# Autodesk Inventor assembly: FO-022
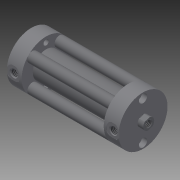
[picture p0: Inventor's stored thumbnail of the model, 180x180]
Saved by Autodesk Inventor 2014 (Build 180170000, 170)
## iProperties
Category: PARTsolutions
Company: BIMBA
Created: 2014-01-19
Part Number: FO-022
Catalog Web Link: www.cadenas.de
Description: FO, FOD, FOR, FOS-Bimba FLAT-1
Vendor: BIMBA
Document SubType Name: Assembly
Designer: Andrew Toennies
Manufacturer: BIMBA
PSOL_IDENT_0: {$CADENAS_DATA\23d-libs\bimba\bimba\bimba_imperial\bimba_full_line\flat_cylinders\fo1\fo1_asmtab.prj
PSOL_IDENT_1: },275 {VTYP=3D},{STYP=ASSTAB},{NB=FO-022},{LINA=FO-022},{NN=FO, FOD, FOR, FOS},{DATE=11.10.2013 12:3
PSOL_IDENT_2: 5:34},{GEOMDATE=17.11.2012 07:08:13},{VERSION=},{LINEID=10},{LINESUBID=-1},{WBVAR=STROKE,ACTING,MNTR
PSOL_IDENT_3: ,MNTF,EE,EEL,B,RT,G,HR,HD,FO,FS,M,PP,TO,S,STPT1,STPT2,STPT3,STPT4,W,Y,RP,CB,TB}  {NB=FO-022},{LINA=F
PSOL_IDENT_4: O-022},{KT=DUMMY},{PN=FO-022},{PNA=(NO ACCESSORIES)},{PNC=FO-022},{BORE=9/16\" (02)},{BORE1=0.562500
PSOL_IDENT_5: 00},{BOREPN=02},{STROKE=2},{STROKEMAX=10.00000000},{ACTING=},{ACTINGALG='','Double Acting, Single En
PSOL_IDENT_6: d Rod [FO]', 'D'  , 'Double Acting, Double End Rod [FOD]', 'R', 'Reverse Acting [FOR]', 'S'  ,'Singl
PSOL_IDENT_7: e Acting [FOS]'},{MNTR=},{MNTF=},{MNT=},{MNTALG='','Standard Counterbored Mounting Holes','1','Pivot
PSOL_IDENT_8: Mount','1N','Pivot Mount 90 Deg. from Standard','3','Threaded Mounting Holes, Both Ends','3F','Thre
PSOL_IDENT_9: aded Mounting Holes, Front','3R','Threaded Mounting Holes, Rear','4','Screw Clearance Holes, Both En
PSOL_IDENT_10: ds','4F','Screw Clearance Holes, Front','4R','Screw Clearance Holes, Rear','5','Nose Mount'},{EEMAX=
PSOL_IDENT_11: 8},{EE=},{EEALG='','Without Extra Extension','EE','With Extra Extension'},{EEL=0.000},{EELALG=0},{B=
PSOL_IDENT_12: },{BALG='','Without Bumper','B','Bumper, Both Ends','BR','Bumper, Rear Only','BF','Bumper, Front Onl
PSOL_IDENT_13: y'},{RT=},{RTALG='', 'Standard Female Thread #8-32',  'MT', 'Male Rod End (Fine) #8-32 [MT]', 'NT'
PSOL_IDENT_14: , 'Non-Threaded Rod (Plain Rod) [NT]'},{G=},{HR=},{HRALG='','N/A'},{HD=},{HDALG='', 'Standard Rear H
PSOL_IDENT_15: ead', 'HD', 'Heavy Duty Rear Head'},{FO=},{FOALG='','N/A'},{FS=},{FSALG='','Standard Friction Seals'
PSOL_IDENT_16: ,'L','Low Friction Seals', 'X', 'Ring Rod Seal'},{FSPNL=},{FSPNX=},{M=},{MALG='','Without Magnet','M'
PSOL_IDENT_17: ,'With Magnet Position 2','M1','With Magnet Position 1','M3','With Magnet Position 3','M4','With Mag
PSOL_IDENT_18: net Position 4'},{PP=},{PPALG='','Standard (ports in line, position #1)'},{TO=},{S=},{SALG='', 'With
PSOL_IDENT_19: out Stainless Steel Fasteners', 'S'  , 'With Stainless Steel Fasteners'},{ST=},{STALG= '' , 'N/A' },
PSOL_IDENT_20: {STPT1=},{STPT1ALG= '' , 'N/A' },{STPT2=},{STPT2ALG= '' , 'N/A' },{STPT3=},{STPT3ALG= '' , 'N/A' },{
PSOL_IDENT_21: STPT4=},{STPT4ALG= '' , 'N/A' },{SOALG='', 'Without Ring Rod Seal', 'X', 'With Ring Rod Seal'},{SO=}
PSOL_IDENT_22: ,{W=},{WALG='', 'Without Wiper', 'W', 'With Wiper'},{Y=},{RP=},{CB=},{TB=},{A=1.12},{BA=0.56},{BA1=0
PSOL_IDENT_23: .56},{BB=0.00},{BB1=0.69},{BC=0.00},{BD=0.00},{B1=0.13},{B11=-},{C=0.88},{DD=2},{D=#4},{CPIL=0.12000
PSOL_IDENT_24: 000},{DC=0.18800000},{DCP=0.12000000},{DCD=0.85500000},{ES=#8-32},{EC=N/A},{ED=0.46},{F=0.25},{H=0.2
PSOL_IDENT_25: 2},{J=0.34},{K=0.14},{K1=0.14},{K2=0.27},{L=#10-32},{ANGLE=45},{LDP=0.20000000},{LP=0.16000000},{LPD
PSOL_IDENT_26: P=0.28000000},{TD=0.65700000},{TDDP=0.10000},{TD1=0.59500},{TD2=0.61000},{TDIN=0.56200},{LSF=0.31250
PSOL_IDENT_27: 000},{LSFDP=0.02000000},{BC1=0.81000},{BC2=1.38000},{BC3=1.96000},{BC4=2.52000},{BD1=1.06000},{BD2=1
PSOL_IDENT_28: .62000},{BD3=2.14000},{BD4=2.70000},{BBB=0.56},{FSADD1=0.25000000},{HDADD1=0.13000000},{MADD1=0.88},
PSOL_IDENT_29: {M1=0.88000000},{M2=0.63000000},{M3=0.38000000},{RL=2.45},{BL=2.08},{LR=1.88},{FSADD=0},{HDADD=0},{M
PSOL_IDENT_30: ADD=0},{ER=},{RL22=0.13},{RL11=0.13000000},{RL1=0.13},{MNTRG=},{MNTRH=},{AC1=0.38000000},{LG1=0.3800
PSOL_IDENT_31: 0000},{LG=0},{RPART=0.08},{AA1=0.06},{AA=-},{AB1=0.75},{AB=-},{AC2=0.00},{AC=-},{AD1=1/2-20},{AD=-},
PSOL_IDENT_32: {AE1=.499/.496},{AE=-},{AF1=0.31},{AF=-},{MM1=0.00000000},{MM=-},{N1=0.00000000},{N=-},{P1=0.0000000
PSOL_IDENT_33: 0},{NB1=0.00000000},{P=-},{R=-},{R1=#4-40},{Q=-},{Q1=0.19},{S1=-},{S2=0.38},{T=-},{T1=0.19},{U=-},{U
PSOL_IDENT_34: 1=0.25},{W1=-},{W11=0.75},{Z=-},{Z1=0.19},{Y1=-},{Y11=0.63},{X=-},{X1=0.17},{DASH=},{RTPN1=},{RTPN2=
PSOL_IDENT_35: },{QPN1=},{QPN2=},{EELPN=},{CBALG='','N/A'},{TBALG='','N/A'},{RPALG='','Without Rod Pivot','RP-1/2','
PSOL_IDENT_36: RP-1/2'},{CBPN=},{TBPN=},{RPPN=},{STPT1PN=},{STPT2PN=},{STPT3PN=},{STPT4PN=},{RPALG1= '' , 'Without
PSOL_IDENT_37: Rod Pivot' , 'F,RP-1/2' , 'RP-1/2 (front)' },{CBALG1='','N/A'},{TBALG1='','N/A'},{CBPN1=},{TBPN1=},{
PSOL_IDENT_38: RPPN1=},{CB1=BC-1},{TB1=-},{RP1=RP-1/2},{LR1=1.88},{PPATH=fo1_asmtpl.prj},{MNTRALG='','Standard Coun
PSOL_IDENT_39: terbored Mounting Holes','1','Pivot Mount','1N','Pivot Mount 90 Deg. from Standard','3R','Threaded M
PSOL_IDENT_40: ounting Holes, Rear','4R','Screw Clearance Holes, Rear'},{MNTFALG='','Standard Counterbored Mounting
PSOL_IDENT_41: Holes','3F','Threaded Mounting Holes, Front','4F','Screw Clearance Holes, Front','5','Nose Mount'},
PSOL_IDENT_42: {MNTPN=},{MNTPNRH=0},{MNTPNRG=0},{WPN=},{HDPN=},{ASSOPTACC=Y},{MATALGHTML=<b>Flat 1 Cylinders:</b><d
PSOL_IDENT_43: l><dt>End Caps & Posts:</dt><dd>- Anodized Aluminum</dd><dt> Seals:</dt><dd>- Buna N </dd><dt>Body:<
PSOL_IDENT_44: /dt><dd>- 304 Stainless Steel</dd><dt>Bearings:</dt><dd>- Oil Impregnated Bronze</dd><dt>Rod:</dt><d
PSOL_IDENT_45: d>-  303 Stainless Steel</dd></dl>}
CNS_NN: FO, FOD, FOR, FOS
CNS_NT: Bimba FLAT-1
CNS_NB: FO-022
CNS_NBSYN: $PNC.
CNS_LINA: FO-022
CNS_PN: FO-022
CNS_PNA: (NO ACCESSORIES)
CNS_PNC: FO-022
CNS_BORE: 9/16" [02]
CNS_BORE1: 0.56250000
CNS_BOREPN: 02
CNS_STROKE: 2.000
CNS_STROKEMAX: 10.00000000
CNS_ACTING: Double Acting, Single End Rod [FO]
CNS_ACTINGALG: '','Double Acting, Single End Rod [FO]', 'D'  , 'Double Acting, Double End Rod [FOD]', 'R', 'Reverse Acting [FOR]', 'S'  ,'Single Acting [FOS]'
CNS_MNTR: Standard Counterbored Mounting Holes
CNS_MNTF: Standard Counterbored Mounting Holes
CNS_MNTALG: '','Standard Counterbored Mounting Holes','1','Pivot Mount','1N','Pivot Mount 90 Deg. from Standard','3','Threaded Mounting Holes, Both Ends','3F','Threaded Mounting Holes, Front','3R','Threaded Mounting Holes, Rear','4','Screw Clearance Holes, Both Ends','4F','Screw Clearance Holes, Front','4R','Screw Clearance Holes, Rear','5','Nose Mount'
CNS_EEMAX: 8.000
CNS_EE: Standard Rod Extension
CNS_EEALG: '','Without Extra Extension','EE','With Extra Extension'
CNS_EEL: 0.000
CNS_EELALG: 0
CNS_B: Without Bumper
CNS_BALG: '','Without Bumper','B','Bumper, Both Ends','BR','Bumper, Rear Only','BF','Bumper, Front Only'
CNS_RT: Standard Female Thread #8-32
CNS_RTALG: '', 'Standard Female Thread #8-32',  'MT', 'Male Rod End (Fine) #8-32 [MT]', 'NT'  , 'Non-Threaded Rod (Plain Rod) [NT]'
CNS_G: Standard Lube
CNS_HR: N/A
CNS_HRALG: '','N/A'
CNS_HD: Standard Rear Head
CNS_HDALG: '', 'Standard Rear Head', 'HD', 'Heavy Duty Rear Head'
CNS_FO: N/A
CNS_FOALG: '','N/A'
CNS_FS: Standard O-Ring Seals
CNS_FSALG: '','Standard Friction Seals','L','Low Friction Seals', 'X', 'Ring Rod Seal'
CNS_M: Without Magnet
CNS_MALG: '','Without Magnet','M','With Magnet Position 2','M1','With Magnet Position 1','M3','With Magnet Position 3','M4','With Magnet Position 4'
CNS_PP: Standard (ports in line, position #1)
CNS_PPALG: '','Standard (ports in line, position #1)'
CNS_TO: Standard -20° to 200°F (-29° to 95°C)
CNS_S: Standard Steel Fasteners
CNS_SALG: '', 'Without Stainless Steel Fasteners', 'S'  , 'With Stainless Steel Fasteners'
CNS_STALG: '' , 'N/A'
CNS_STPT1: N/A
CNS_STPT1ALG: '' , 'N/A'
CNS_STPT2: N/A
CNS_STPT2ALG: '' , 'N/A'
CNS_STPT3: N/A
CNS_STPT3ALG: '' , 'N/A'
CNS_STPT4: N/A
CNS_STPT4ALG: '' , 'N/A'
CNS_SOALG: '', 'Without Ring Rod Seal', 'X', 'With Ring Rod Seal'
CNS_W: Without Wiper
CNS_WALG: '', 'Without Wiper', 'W', 'With Wiper'
CNS_Y: Non-Coated (Standard)
CNS_RP: Without Rod Pivot
CNS_CB: N/A
CNS_TB: N/A
CNS_A: 1.12
CNS_BA: 0.56
CNS_BA1: 0.56
CNS_BB: 0.00
CNS_BB1: 0.69
CNS_BC: 0.00
CNS_BD: 0.00
CNS_B1: 0.13
CNS_B11: -
CNS_C: 0.88
CNS_DD: 2
CNS_D: #4
CNS_CPIL: 0.12000000
CNS_DC: 0.18800000
CNS_DCP: 0.12000000
CNS_DCD: 0.85500000
CNS_ES: #8-32
CNS_EC: N/A
CNS_ED: 0.46
CNS_F: 0.25
CNS_H: 0.22
CNS_J: 0.34
CNS_K: 0.14
CNS_K1: 0.14
CNS_K2: 0.27
CNS_L: #10-32
CNS_ANGLE: 45
CNS_LDP: 0.20000000
CNS_LP: 0.16000000
CNS_LPDP: 0.28000000
CNS_TD: 0.65700000
CNS_TDDP: 0.10000
CNS_TD1: 0.59500
CNS_TD2: 0.61000
CNS_TDIN: 0.56200
CNS_LSF: 0.31250000
CNS_LSFDP: 0.02000000
CNS_BC1: 0.81000
CNS_BC2: 1.38000
CNS_BC3: 1.96000
CNS_BC4: 2.52000
CNS_BD1: 1.06000
CNS_BD2: 1.62000
CNS_BD3: 2.14000
CNS_BD4: 2.70000
CNS_BBB: 0.560
CNS_FSADD1: 0.25000000
CNS_HDADD1: 0.13000000
CNS_MADD1: 0.880
CNS_M1: 0.88000000
CNS_M2: 0.63000000
CNS_M3: 0.38000000
CNS_RL: 2.450
CNS_BL: 2.080
CNS_LR: 1.880
CNS_FSADD: 0.000
CNS_HDADD: 0.000
CNS_MADD: 0.000
CNS_RL22: 0.130
CNS_RL11: 0.13000000
CNS_RL1: 0.130
CNS_AC1: 0.38000000
CNS_LG1: 0.38000000
CNS_LG: 0.000
CNS_RPART: 0.080
CNS_AA1: 0.06
CNS_AA: -
CNS_AB1: 0.75
CNS_AB: -
CNS_AC2: 0.00
CNS_AC: -
CNS_AD1: 1/2-20
CNS_AD: -
CNS_AE1: .499/.496
CNS_AE: -
CNS_AF1: 0.31
CNS_AF: -
CNS_MM1: 0.00000000
CNS_MM: -
CNS_N1: 0.00000000
CNS_N: -
CNS_P1: 0.00000000
CNS_NB1: 0.00000000
CNS_P: -
CNS_R: -
CNS_R1: #4-40
CNS_Q: -
CNS_Q1: 0.19
CNS_S1: -
CNS_S2: 0.38
CNS_T: -
CNS_T1: 0.19
CNS_U: -
CNS_U1: 0.25
CNS_W1: -
CNS_W11: 0.75
CNS_Z: -
CNS_Z1: 0.19
CNS_Y1: -
CNS_Y11: 0.63
CNS_X: -
CNS_X1: 0.17
CNS_CBALG: '','N/A'
CNS_TBALG: '','N/A'
CNS_RPALG: '','Without Rod Pivot','RP-1/2','RP-1/2'
CNS_RPALG1: '' , 'Without Rod Pivot' , 'F,RP-1/2' , 'RP-1/2 (front)'
CNS_CBALG1: '','N/A'
CNS_TBALG1: '','N/A'
CNS_CB1: BC-1
CNS_TB1: -
CNS_RP1: RP-1/2
CNS_LR1: 1.880
CNS_PPATH: fo1_asmtpl.prj
CNS_MNTRALG: '','Standard Counterbored Mounting Holes','1','Pivot Mount','1N','Pivot Mount 90 Deg. from Standard','3R','Threaded Mounting Holes, Rear','4R','Screw Clearance Holes, Rear'
CNS_MNTFALG: '','Standard Counterbored Mounting Holes','3F','Threaded Mounting Holes, Front','4F','Screw Clearance Holes, Front','5','Nose Mount'
CNS_MNTPNRH: 0
CNS_MNTPNRG: 0
CNS_ASSOPTACC: Y
CNS_MATALGHTML: <b>Flat 1 Cylinders:</b><dl><dt>End Caps & Posts:</dt><dd>- Anodized Aluminum</dd><dt> Seals:</dt><dd>- Buna N </dd><dt>Body:</dt><dd>- 304 Stainless Steel</dd><dt>Bearings:</dt><dd>- Oil Impregnated Bronze</dd><dt>Rod:</dt><dd>-  303 Stainless Steel</dd></dl>
SUPPLIER: BIMBA
ARTICLENO: FO-022
BOMINFO: FO-022
CREATOR: CADENAS GmbH
Title: FO-022
Author: Cadenas PARTsolutions
Comments: Bimba FLAT-1
## Documents named in this file (7)
- C:\Users\Andrew Toennies\Documents\GitHub\2014buildCAD\New Shooter\0.5625 in bore 2 in stroke compact cylinder - BIMBA\FO-022.iam
- C:\Users\Andrew Toennies\Documents\GitHub\2014buildCAD\New Shooter\0.5625 in bore 2 in stroke compact cylinder - BIMBA\02-2-0_13-FO1_BM_heads.ipt
- C:\Users\Andrew Toennies\Documents\GitHub\2014buildCAD\New Shooter\0.5625 in bore 2 in stroke compact cylinder - BIMBA\022_08-FO1_BM_tube.ipt
- C:\Users\Andrew Toennies\Documents\GitHub\2014buildCAD\New Shooter\0.5625 in bore 2 in stroke compact cylinder - BIMBA\02-1-0_13-FO1_BM_heads.ipt
- C:\Users\Andrew Toennies\Documents\GitHub\2014buildCAD\New Shooter\0.5625 in bore 2 in stroke compact cylinder - BIMBA\022_452_45-FO1_BM_rod.ipt
- C:\Users\Andrew Toennies\Documents\GitHub\2014buildCAD\New Shooter\0.5625 in bore 2 in stroke compact cylinder - BIMBA\0_56250_0800000000000001-rod_part.ipt
- C:\Users\Andrew Toennies\Documents\GitHub\2014buildCAD\New Shooter\0.5625 in bore 2 in stroke compact cylinder - BIMBA\022_08-FO1_BM_r.ipt
## Components (9 placed, 6 different names)
1. 02-2-0_13-FO1_BM_heads:1 — Insert:1, Insert:2, Insert:3, Insert:4, Mate:3
2. 022_08-FO1_BM_tube:1 — Flush:1, Mate:1, Mate:2
3. 02-1-0_13-FO1_BM_heads:1 — Insert:5, Insert:6, Mate:2
4. 022_452_45-FO1_BM_rod:1 — Insert:7, Mate:3
5. 0_56250_0800000000000001-rod_part:1 — Insert:7, Mate:1
6. 022_08-FO1_BM_r:1 — Insert:1, Insert:6
7. 022_08-FO1_BM_r:2 — Insert:4
8. 022_08-FO1_BM_r:3 — Insert:3, Insert:5, Flush:1
9. 022_08-FO1_BM_r:4 — Insert:2
## Relationships (11: Insert 7, Mate 3, Flush 1)
- Insert:1: 02-2-0_13-FO1_BM_heads:1 ↔ 022_08-FO1_BM_r:1
- Insert:2: 02-2-0_13-FO1_BM_heads:1 ↔ 022_08-FO1_BM_r:4
- Insert:3: 02-2-0_13-FO1_BM_heads:1 ↔ 022_08-FO1_BM_r:3
- Insert:4: 02-2-0_13-FO1_BM_heads:1 ↔ 022_08-FO1_BM_r:2
- Insert:5: 02-1-0_13-FO1_BM_heads:1 ↔ 022_08-FO1_BM_r:3
- Insert:6: 02-1-0_13-FO1_BM_heads:1 ↔ 022_08-FO1_BM_r:1
- Insert:7: 022_452_45-FO1_BM_rod:1 ↔ 0_56250_0800000000000001-rod_part:1
- Flush:1: 022_08-FO1_BM_tube:1 ↔ 022_08-FO1_BM_r:3
- Mate:1: 022_08-FO1_BM_tube:1 ↔ 0_56250_0800000000000001-rod_part:1
- Mate:2: 022_08-FO1_BM_tube:1 ↔ 02-1-0_13-FO1_BM_heads:1
- Mate:3: 02-2-0_13-FO1_BM_heads:1 ↔ 022_452_45-FO1_BM_rod:1
